# Autodesk Inventor assembly: Head
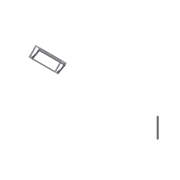
[picture p0: Inventor's stored thumbnail of the model, 180x180]
Saved by Autodesk Inventor 2014 SP1 (Build 180222100, 222)
## iProperties
Created: 2015-02-11
Part Number: Head
Document SubType Name: Assembly
Designer: Simen
Author: Simen
## Documents named in this file (11)
- C:\Users\Simen\Documents\git\Eit\skjellet\Head2.iam
- C:\Users\Simen\Documents\git\Eit\skjellet\HBL45TS6hbl45ts6.ipt
- C:\Users\Simen\Documents\git\Eit\skjellet\HBL135TS6.iam
- C:\Users\Simen\Documents\git\Eit\skjellet\KHFS5_2020_386.ipt
- C:\Users\Simen\Documents\git\Eit\skjellet\KHFS5_2020_391.ipt
- C:\Users\Simen\Documents\git\Eit\skjellet\HBLFSN5.iam
- C:\Users\Simen\Documents\git\Eit\skjellet\KHFS5_2020_220.ipt
- C:\Users\Simen\Documents\git\Eit\skjellet\KHFS5_2020_195,5.ipt
- C:\Users\Simen\Documents\git\Eit\skjellet\KHFS5_2020_234,5.ipt
- C:\Users\Simen\Documents\git\Eit\skjellet\frontPlate_half.ipt
- C:\Users\Simen\Documents\git\Eit\skjellet\KHFS5_2020_60.ipt
## Components (18 placed, 5 different names)
1. HBL45TS6hbl45ts6:2 — Mate:41, Flush:39, Mate:44, Mate:74, Mate:75, Flush:59
2. HBL135TS6:2 [sub-assembly] — Mate:73, Flush:60, Mate:76
3. KHFS5-2020-4000:17 — Flush:64, Mate:83, Flush:65, Flush:66, Flush:67, Flush:68, Mate:84, Flush:83
4. KHFS5-2020-4000:18 — Mate:41, Flush:39, Mate:44, Flush:76
5. KHFS5-2020-4000:19 — Flush:58, Mate:81, Flush:63, Mate:82, Flush:71, Mate:90
6. KHFS5-2020-4000:27 — Flush:58, Flush:69, Flush:70, Flush:74, Flush:75
7. HBLFSN5:1 [sub-assembly] — Flush:72, Mate:85, Mate:88
8. KHFS5-2020-4000:34 — Mate:73, Mate:74, Mate:75, Flush:59, Flush:60, Mate:76, Flush:64, Flush:67, Flush:68, Mate:84, Flush:82
9. HBL45TS6hbl45ts6:3 — Mate:81, Flush:63
10. HBL135TS6:3 [sub-assembly] — Mate:86, Flush:73
11. KHFS5-2020-4000:35 — Mate:82, Mate:83, Flush:65, Flush:66, Mate:93
12. KHFS5-2020-4000:36 — Flush:69, Flush:70, Flush:71, Flush:72, Mate:85, Mate:87, Mate:90
13. KHFS5-2020-4000:37 — Mate:86, Mate:87, Flush:73, Mate:88, Flush:81, Mate:92
14. KHFS5-2020-4000:38 — Flush:74, Flush:75, Flush:76, Flush:77, Flush:78
15. KHFS5-2020-4000:39 — Flush:77, Flush:78
16. frontPlate_half:1 — Mate:93, Flush:82, Flush:83
17. KHFS5-2020-4000:40 — Flush:81, Mate:92
18. KHFS5-2020-4000:41
## Relationships (47: Flush 25, Mate 22)
- Mate:41: HBL45TS6hbl45ts6:2 ↔ KHFS5-2020-4000:18
- Flush:39: HBL45TS6hbl45ts6:2 ↔ KHFS5-2020-4000:18
- Mate:44: HBL45TS6hbl45ts6:2 ↔ KHFS5-2020-4000:18
- Flush:58: KHFS5-2020-4000:19 ↔ KHFS5-2020-4000:27
- Mate:73: HBL135TS6:2 ↔ KHFS5-2020-4000:34
- Mate:74: HBL45TS6hbl45ts6:2 ↔ KHFS5-2020-4000:34
- Mate:75: HBL45TS6hbl45ts6:2 ↔ KHFS5-2020-4000:34
- Flush:59: HBL45TS6hbl45ts6:2 ↔ KHFS5-2020-4000:34
- Flush:60: HBL135TS6:2 ↔ KHFS5-2020-4000:34
- Mate:76: HBL135TS6:2 ↔ KHFS5-2020-4000:34
- [Mate]: HBL135TS6:3 ↔ KHFS5-2020-4000:35
- [Mate]: HBL45TS6hbl45ts6:3 ↔ KHFS5-2020-4000:35
- [Mate]: HBL45TS6hbl45ts6:3 ↔ KHFS5-2020-4000:35
- [Flush]: HBL45TS6hbl45ts6:3 ↔ KHFS5-2020-4000:35
- [Flush]: HBL135TS6:3 ↔ KHFS5-2020-4000:35
- [Mate]: HBL135TS6:3 ↔ KHFS5-2020-4000:35
- Mate:81: KHFS5-2020-4000:19 ↔ HBL45TS6hbl45ts6:3
- Flush:63: KHFS5-2020-4000:19 ↔ HBL45TS6hbl45ts6:3
- Mate:82: KHFS5-2020-4000:19 ↔ KHFS5-2020-4000:35
- Flush:64: KHFS5-2020-4000:17 ↔ KHFS5-2020-4000:34
- Mate:83: KHFS5-2020-4000:17 ↔ KHFS5-2020-4000:35
- Flush:65: KHFS5-2020-4000:17 ↔ KHFS5-2020-4000:35
- Flush:66: KHFS5-2020-4000:17 ↔ KHFS5-2020-4000:35
- Flush:67: KHFS5-2020-4000:17 ↔ KHFS5-2020-4000:34
- Flush:68: KHFS5-2020-4000:17 ↔ KHFS5-2020-4000:34
- Mate:84: KHFS5-2020-4000:17 ↔ KHFS5-2020-4000:34
- Flush:69: KHFS5-2020-4000:27 ↔ KHFS5-2020-4000:36
- Flush:70: KHFS5-2020-4000:27 ↔ KHFS5-2020-4000:36
- Flush:71: KHFS5-2020-4000:19 ↔ KHFS5-2020-4000:36
- Flush:72: HBLFSN5:1 ↔ KHFS5-2020-4000:36
- Mate:85: HBLFSN5:1 ↔ KHFS5-2020-4000:36
- Mate:86: HBL135TS6:3 ↔ KHFS5-2020-4000:37
- Mate:87: KHFS5-2020-4000:36 ↔ KHFS5-2020-4000:37
- Flush:73: HBL135TS6:3 ↔ KHFS5-2020-4000:37
- Mate:88: HBLFSN5:1 ↔ KHFS5-2020-4000:37
- [Mate]: KHFS5-2020-4000:38 ↔ KHFS5-2020-4000:39
- Flush:74: KHFS5-2020-4000:27 ↔ KHFS5-2020-4000:38
- Flush:75: KHFS5-2020-4000:27 ↔ KHFS5-2020-4000:38
- Flush:76: KHFS5-2020-4000:18 ↔ KHFS5-2020-4000:38
- Flush:77: KHFS5-2020-4000:38 ↔ KHFS5-2020-4000:39
- Flush:78: KHFS5-2020-4000:38 ↔ KHFS5-2020-4000:39
- Mate:90: KHFS5-2020-4000:19 ↔ KHFS5-2020-4000:36
- Flush:81: KHFS5-2020-4000:37 ↔ KHFS5-2020-4000:40
- Mate:92: KHFS5-2020-4000:37 ↔ KHFS5-2020-4000:40
- Mate:93: KHFS5-2020-4000:35 ↔ frontPlate_half:1
- Flush:82: KHFS5-2020-4000:34 ↔ frontPlate_half:1
- Flush:83: KHFS5-2020-4000:17 ↔ frontPlate_half:1
## Named parameters: d170_d162 = 0 mm, d171_d163 = 0 mm, d172_d164 = 0 mm, d173_d165 = 0 mm, d174_d166 = 0 mm, d175_d168 = 0 mm, d215_d212 = 0 mm
